# Autodesk Inventor assembly: Regulator
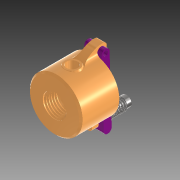
[picture p0: Inventor's stored thumbnail of the model, 180x180]
Saved by Autodesk Inventor 2020 (Build 240168000, 168)
## iProperties
Created: 2021-05-21
Part Number: Regulator
Document SubType Name: Assembly
Designer: DDeGo
Author: DDeGo
## Documents named in this file (10)
- C:\Users\DDeGo\Documents\Drew\Projects\AirWankelEngine\cad\MiniRegulator\Regulator.iam
- C:\Users\DDeGo\Documents\Drew\Projects\AirWankelEngine\cad\MiniRegulator\RegulatorBody.ipt
- C:\Users\DDeGo\Documents\Drew\Projects\AirWankelEngine\cad\MiniRegulator\RegulatorValve.ipt
- C:\Users\DDeGo\Documents\Drew\Projects\AirWankelEngine\cad\hardware\6mm bb.ipt
- C:\Users\DDeGo\Documents\Drew\Projects\AirWankelEngine\cad\hardware\oring_4x8.ipt
- C:\Users\DDeGo\Documents\Drew\Projects\AirWankelEngine\cad\MiniRegulator\RegulatorRubberSheet.ipt
- C:\Users\DDeGo\Documents\Drew\Projects\AirWankelEngine\cad\MiniRegulator\RegulatorHinge.ipt
- C:\Users\DDeGo\Documents\Drew\Projects\AirWankelEngine\cad\MiniRegulator\M3x30 SHCS.ipt
- C:\Users\DDeGo\Documents\Drew\Projects\AirWankelEngine\cad\MiniRegulator\Spring.ipt
- C:\Users\DDeGo\Documents\Drew\Projects\AirWankelEngine\cad\MiniRegulator\RegulatorBaffleCap.ipt
## Components (9 placed, 9 different names)
1. RegulatorBody:1 — Mate:1, Mate:2, Mate:6, Mate:8, Tangent:1, Mate:10, Mate:11, Mate:13, Flush:1, Mate:14, Mate:15
2. RegulatorValve:1 — Mate:10, Mate:12, Tangent:2, Mate:14
3. 6mm bb:1 — Mate:1, Tangent:2
4. oring_4x8:1 — Mate:2, Tangent:1
5. RegulatorRubberSheet:1 — Mate:11, Mate:12, Tangent:3
6. RegulatorHinge:1 — Mate:6, Tangent:3, Mate:15
7. M3x30 SHCS:1 — Mate:8, Mate:9
8. Spring:1 — Mate:9
9. RegulatorBaffleCap:1 — Mate:13, Flush:1
## Relationships (15: Mate 11, Tangent 3, Flush 1)
- Mate:1: RegulatorBody:1 ↔ 6mm bb:1
- Mate:2: RegulatorBody:1 ↔ oring_4x8:1
- Mate:6: RegulatorBody:1 ↔ RegulatorHinge:1
- Mate:8: RegulatorBody:1 ↔ M3x30 SHCS:1
- Mate:9: M3x30 SHCS:1 ↔ Spring:1
- Tangent:1: RegulatorBody:1 ↔ oring_4x8:1
- Mate:10: RegulatorBody:1 ↔ RegulatorValve:1
- Mate:11: RegulatorBody:1 ↔ RegulatorRubberSheet:1
- Mate:12: RegulatorValve:1 ↔ RegulatorRubberSheet:1
- Mate:13: RegulatorBody:1 ↔ RegulatorBaffleCap:1
- Flush:1: RegulatorBody:1 ↔ RegulatorBaffleCap:1
- Tangent:2: RegulatorValve:1 ↔ 6mm bb:1
- Tangent:3: RegulatorRubberSheet:1 ↔ RegulatorHinge:1
- Mate:14: RegulatorBody:1 ↔ RegulatorValve:1
- Mate:15 (0.15 mm): RegulatorBody:1 ↔ RegulatorHinge:1
